# Autodesk Inventor assembly: AssemblyFidget
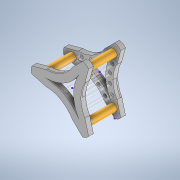
[picture p0: Inventor's stored thumbnail of the model, 180x180]
Saved by Autodesk Inventor 2022.4 (Build 264492010, 492A)
## iProperties
Created: 2023-09-20
Part Number: AssemblyFidget
Document SubType Name: Assembly
Designer: tmass
Author: tmass
## Documents named in this file (4)
- C:\Users\tmass\OneDrive\Bureau\UFO paper\3D models\Fidget\Inventor\AssemblyCoil.iam
- C:\Users\tmass\OneDrive\Bureau\UFO paper\3D models\Fidget\Inventor\Coil holder.ipt
- C:\Users\tmass\OneDrive\Bureau\UFO paper\3D models\Fidget\Inventor\Brass pillar.ipt
- C:\Users\tmass\OneDrive\Bureau\UFO paper\3D models\Fidget\Inventor\Plastic pillars.ipt
## Components (17 placed, 3 different names)
1. Coil holder:1 — Mate:22, Mate:23, Mate:24, Mate:25, Mate:26, Mate:27, Mate:28, Mate:29, Mate:30, Mate:31, Mate:32, Mate:33, Mate:34, Mate:35, Mate:36, Mate:37, Mate:38, Mate:39, Mate:40, Mate:41, Mate:42, Mate:43, Mate:44, Mate:45, Mate:46, Mate:47, Mate:48, Mate:49, Mate:50, Mate:51, Mate:52
2. Brass pillar:1 — Mate:25, Mate:27, Mate:53, Mate:54
3. Brass pillar:2 — Mate:23, Mate:26
4. Brass pillar:3 — Mate:24, Mate:28, Mate:55
5. Plastic pillars:1 — Mate:39, Mate:40
6. Plastic pillars:2 — Mate:47, Mate:48
7. Plastic pillars:3 — Mate:51, Mate:52
8. Plastic pillars:4 — Mate:45, Mate:46
9. Plastic pillars:5 — Mate:43, Mate:44
10. Plastic pillars:6 — Mate:41, Mate:42
11. Plastic pillars:7 — Mate:35, Mate:36
12. Plastic pillars:8 — Mate:31, Mate:32
13. Plastic pillars:9 — Mate:33, Mate:34
14. Plastic pillars:10 — Mate:37, Mate:38
15. Plastic pillars:11 — Mate:29, Mate:30
16. Plastic pillars:12 — Mate:49, Mate:50
17. Coil holder:2 — Mate:53, Mate:54, Mate:55
## Relationships (35: Mate 34, Angle 1)
- Mate:22: Coil holder:1
- Angle:1 (0 deg)
- Mate:23: Coil holder:1 ↔ Brass pillar:2
- Mate:24: Coil holder:1 ↔ Brass pillar:3
- Mate:25: Coil holder:1 ↔ Brass pillar:1
- Mate:26: Coil holder:1 ↔ Brass pillar:2
- Mate:27: Coil holder:1 ↔ Brass pillar:1
- Mate:28: Coil holder:1 ↔ Brass pillar:3
- Mate:29: Coil holder:1 ↔ Plastic pillars:11
- Mate:30: Coil holder:1 ↔ Plastic pillars:11
- Mate:31: Coil holder:1 ↔ Plastic pillars:8
- Mate:32: Coil holder:1 ↔ Plastic pillars:8
- Mate:33: Coil holder:1 ↔ Plastic pillars:9
- Mate:34: Coil holder:1 ↔ Plastic pillars:9
- Mate:35: Coil holder:1 ↔ Plastic pillars:7
- Mate:36: Coil holder:1 ↔ Plastic pillars:7
- Mate:37: Coil holder:1 ↔ Plastic pillars:10
- Mate:38: Coil holder:1 ↔ Plastic pillars:10
- Mate:39: Coil holder:1 ↔ Plastic pillars:1
- Mate:40: Coil holder:1 ↔ Plastic pillars:1
- Mate:41: Coil holder:1 ↔ Plastic pillars:6
- Mate:42: Coil holder:1 ↔ Plastic pillars:6
- Mate:43: Coil holder:1 ↔ Plastic pillars:5
- Mate:44: Coil holder:1 ↔ Plastic pillars:5
- Mate:45: Coil holder:1 ↔ Plastic pillars:4
- Mate:46: Coil holder:1 ↔ Plastic pillars:4
- Mate:47: Coil holder:1 ↔ Plastic pillars:2
- Mate:48: Coil holder:1 ↔ Plastic pillars:2
- Mate:49: Coil holder:1 ↔ Plastic pillars:12
- Mate:50: Coil holder:1 ↔ Plastic pillars:12
- Mate:51: Coil holder:1 ↔ Plastic pillars:3
- Mate:52: Coil holder:1 ↔ Plastic pillars:3
- Mate:53: Brass pillar:1 ↔ Coil holder:2
- Mate:54: Brass pillar:1 ↔ Coil holder:2
- Mate:55: Brass pillar:3 ↔ Coil holder:2
